# Autodesk Inventor assembly: ASY МОО 001 отстойник осветлитель
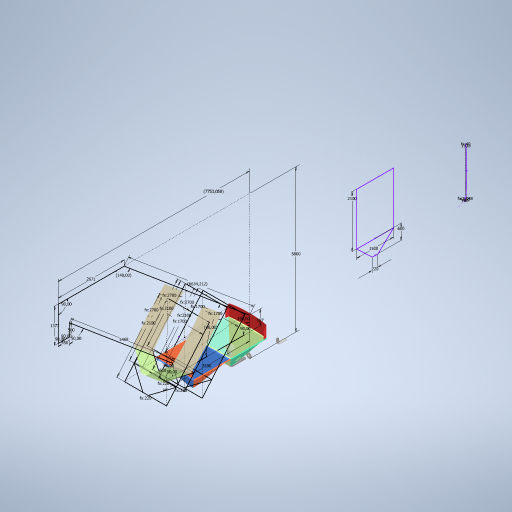
[picture p0: Inventor's stored thumbnail of the model, 512x512]
Saved by Autodesk Inventor 2024.2 (Build 282272000, 272)
## iProperties
Created: 2024-04-28
Part Number: ASY МОО 001 отстойник осветлитель
Document SubType Name: Weldment
Designer: admin
Weld Material: Welded Aluminum-6061
Mass: 420020 g
Surface Area: 719213 cm^2
Volume: 106788 cm^3
Density: 3.93322 g/cm^3
Author: admin
## Documents named in this file (20)
- C:\Users\admin\YandexDisk-badmisterfox\домашниий пк\Inventor\Manturovo\Manturovo_Se-clar\ASY МОО 001 отстойник осветлитель.iam
- C:\Users\admin\YandexDisk-badmisterfox\домашниий пк\Inventor\Manturovo\Manturovo_Se-clar\МОО 020 лист борт 1.ipt
- C:\Users\admin\YandexDisk-badmisterfox\домашниий пк\Inventor\Manturovo\Manturovo_Se-clar\МОО 010 лист спина 1.ipt
- C:\Users\admin\YandexDisk-badmisterfox\домашниий пк\Inventor\Manturovo\Manturovo_Se-clar\Пример емкости.ipt
- C:\Users\admin\YandexDisk-badmisterfox\домашниий пк\Inventor\Manturovo\Manturovo_Se-clar\МОО 030 лист брюхо 1.ipt
- C:\Users\admin\YandexDisk-badmisterfox\домашниий пк\Inventor\Manturovo\Manturovo_Se-clar\МОО 040 шпангоут борт 1.ipt
- C:\Users\admin\YandexDisk-badmisterfox\домашниий пк\Inventor\Manturovo\Manturovo_Se-clar\МОО 041 шпангоут спина 1.ipt
- C:\Users\admin\YandexDisk-badmisterfox\домашниий пк\Inventor\Manturovo\Manturovo_Se-clar\МОО 050 стрингер спина 1.ipt
- C:\Users\admin\YandexDisk-badmisterfox\домашниий пк\Inventor\Manturovo\Manturovo_Se-clar\Рама основания\ASY МОО 040 рама основания.iam
- C:\Users\admin\YandexDisk-badmisterfox\домашниий пк\Inventor\Manturovo\Manturovo_Se-clar\ASY МОО 060 ракета.iam
- C:\Users\admin\YandexDisk-badmisterfox\домашниий пк\Inventor\Manturovo\Manturovo_Se-clar\Content Center Files\en-US\ISO 5251 B 3D\ISO 5251 Bends 3D without straight ends(90 deg) DN80 2 2.ipt
- C:\Users\admin\YandexDisk-badmisterfox\домашниий пк\Inventor\Manturovo\Manturovo_Se-clar\Content Center Files\en-US\ISO 5251(1)\ISO 5251 Concentric reducers DN80 x DN65 3,2 3,2.ipt
- C:\Users\admin\YandexDisk-badmisterfox\домашниий пк\Inventor\Manturovo\Manturovo_Se-clar\ASY МОО 020 конус.iam
- C:\Users\admin\YandexDisk-badmisterfox\домашниий пк\Inventor\Manturovo\Manturovo_Se-clar\ракета\МОО 064 ракета труба.ipt
- C:\Users\admin\YandexDisk-badmisterfox\домашниий пк\Inventor\Manturovo\Manturovo_Se-clar\х_размеры МОО отстойник осветлитель Dummu.ipt
- C:\Users\admin\YandexDisk-badmisterfox\домашниий пк\Inventor\Manturovo\Manturovo_Se-clar\МОО 012 лист спина 2.ipt
- C:\Users\admin\YandexDisk-badmisterfox\домашниий пк\Inventor\Manturovo\Manturovo_Se-clar\ракета\МОО 065 ракета труба 5.ipt
- C:\Users\admin\YandexDisk-badmisterfox\домашниий пк\Inventor\Manturovo\Manturovo_Se-clar\ракета\МОО 066 ракета труба 6.ipt
- C:\Users\admin\YandexDisk-badmisterfox\домашниий пк\Inventor\Manturovo\Manturovo_Se-clar\ракета\МОО 067 ракета труба 7.ipt
- C:\Users\admin\YandexDisk-badmisterfox\домашниий пк\Inventor\Manturovo\Manturovo_Se-clar\Content Center Files\en-US\DIN EN 1092-1 01 - PN 25\DIN EN 1092-1 Plate Flange for Welding Type 01 - PN 25 80 x 88.9.ipt
## Components (52 placed, 19 different names)
1. Пример емкости:1 — Mate:1, Mate:2, Mate:3, Mate:4, Flush:2
2. х_размеры МОО отстойник осветлитель Dummu:1
3. ASY МОО 040 рама основания:1 [sub-assembly] — Flush:19, Flush:20, Flush:21
4. МОО 020 лист борт 1:2 — Flush:6, Angle:1, Symmetry:1, Mate:5, Mate:8
5. МОО 010 лист спина 1:1 — Flush:1, Mate:3, Mate:4, Flush:3, Flush:6, Mate:7, Mate:8, Mate:10
6. МОО 020 лист борт 1:1 — Flush:1, Symmetry:1, Mate:6, Flush:7, Mate:7, Mate:10, Flush:8, Flush:9, Flush:13
7. МОО 030 лист брюхо 1:1 — Mate:5, Mate:6, Flush:7, Mate:9
8. ASY МОО 060 ракета:1 [sub-assembly] — Flush:23, Rigid:10
9. ISO 5251 Bends 3D without straight ends(90 deg) DN80 2:1 — Rigid:2, Rigid:3
10. ISO 5251 Concentric reducers DN80 x DN65 3,2:1 — Rigid:2, Rigid:10
11. ASY МОО 020 конус:1 [sub-assembly] — Flush:22, Mate:16, Tangent:1, Flush:28
12. МОО 064 ракета труба:1 — Rigid:3, Cylindrical:1
13. МОО 010 лист спина 1:2
14. МОО 010 лист спина 1:3 — Flush:24
15. МОО 012 лист спина 2:1 — Mate:15, Mate:16, Tangent:1, Flush:27
16. МОО 065 ракета труба 5:1 — Rigid:5
17. МОО 066 ракета труба 6:1 — Rigid:5, Rigid:6
18. МОО 067 ракета труба 7:1 — Rigid:6, Rigid:7
19. DIN EN 1092-1 Plate Flange for Welding Type 01 - PN 25 80 x 88.9:1 — Flush:25, Flush:26, Mate:18, Cylindrical:1
20. ISO 5251 Concentric reducers DN80 x DN65 3,2:2 — Rigid:7
21. МОО 040 шпангоут борт 1:1 — Flush:8, Flush:9, Flush:10, Symmetry:2, Flush:11, Mate:11, Flush:14
22. МОО 041 шпангоут спина 1:2 — Mate:11, Flush:12
23. МОО 040 шпангоут борт 1:2 — Flush:10, Symmetry:2, Flush:11, Flush:15, Flush:16
24. МОО 040 шпангоут борт 1:3
25. МОО 041 шпангоут спина 1:3
26. МОО 040 шпангоут борт 1:4
27. МОО 040 шпангоут борт 1:5
28. МОО 041 шпангоут спина 1:4
29. МОО 040 шпангоут борт 1:6
30. МОО 040 шпангоут борт 1:7
31. МОО 041 шпангоут спина 1:5
32. МОО 040 шпангоут борт 1:8
33. МОО 040 шпангоут борт 1:9
34. МОО 041 шпангоут спина 1:6
35. МОО 040 шпангоут борт 1:10
36. МОО 040 шпангоут борт 1:11
37. МОО 041 шпангоут спина 1:7
38. МОО 040 шпангоут борт 1:12
39. МОО 040 шпангоут борт 1:13
40. МОО 041 шпангоут спина 1:8
41. МОО 040 шпангоут борт 1:14
42. МОО 040 шпангоут борт 1:15
43. МОО 041 шпангоут спина 1:9
44. МОО 040 шпангоут борт 1:16
45. МОО 050 стрингер спина 1:1 — Flush:13, Flush:14, Flush:17
46. МОО 050 стрингер спина 1:2 — Flush:15, Flush:16, Flush:17
47. МОО 050 стрингер спина 1:3
48. МОО 050 стрингер спина 1:4
49. МОО 050 стрингер спина 1:5
50. МОО 050 стрингер спина 1:6
51. МОО 050 стрингер спина 1:7
52. МОО 050 стрингер спина 1:8
## Component patterns: (8 elements, first: МОО 040 шпангоут борт 1:1 + МОО 041 шпангоут спина 1:2 + МОО 040 шпангоут борт 1:2), (4 elements, first: МОО 050 стрингер спина 1:1 + МОО 050 стрингер спина 1:2)
## Relationships (50: Flush 25, Mate 14, WeldJoint 6, Symmetry 2, Angle 1, Tangent 1, CylindricalJoint 1)
- Flush:1: МОО 010 лист спина 1:1 ↔ МОО 020 лист борт 1:1
- Mate:1: Пример емкости:1
- Mate:2: Пример емкости:1
- Mate:3: Пример емкости:1 ↔ МОО 010 лист спина 1:1
- Mate:4: Пример емкости:1 ↔ МОО 010 лист спина 1:1
- Flush:2: Пример емкости:1
- Flush:3: МОО 010 лист спина 1:1
- Flush:6: МОО 020 лист борт 1:2 ↔ МОО 010 лист спина 1:1
- Angle:1 (180 deg): МОО 020 лист борт 1:2
- Symmetry:1: МОО 020 лист борт 1:2 ↔ МОО 020 лист борт 1:1
- Mate:5: МОО 020 лист борт 1:2 ↔ МОО 030 лист брюхо 1:1
- Mate:6: МОО 020 лист борт 1:1 ↔ МОО 030 лист брюхо 1:1
- Flush:7: МОО 020 лист борт 1:1 ↔ МОО 030 лист брюхо 1:1
- Mate:7: МОО 010 лист спина 1:1 ↔ МОО 020 лист борт 1:1
- Mate:8: МОО 020 лист борт 1:2 ↔ МОО 010 лист спина 1:1
- Mate:9: МОО 030 лист брюхо 1:1
- Mate:10 (-20 mm): МОО 010 лист спина 1:1 ↔ МОО 020 лист борт 1:1
- Flush:8: МОО 020 лист борт 1:1 ↔ МОО 040 шпангоут борт 1:1
- Flush:9 (250 mm): МОО 020 лист борт 1:1 ↔ МОО 040 шпангоут борт 1:1
- Flush:10: МОО 040 шпангоут борт 1:1 ↔ МОО 040 шпангоут борт 1:2
- Symmetry:2: МОО 040 шпангоут борт 1:1 ↔ МОО 040 шпангоут борт 1:2
- Flush:11: МОО 040 шпангоут борт 1:1 ↔ МОО 040 шпангоут борт 1:2
- Mate:11: МОО 040 шпангоут борт 1:1 ↔ МОО 041 шпангоут спина 1:2
- Flush:12: МОО 041 шпангоут спина 1:2
- Flush:13: МОО 020 лист борт 1:1 ↔ МОО 050 стрингер спина 1:1
- Flush:14 (3 mm): МОО 040 шпангоут борт 1:1 ↔ МОО 050 стрингер спина 1:1
- Flush:15 (-250 mm): МОО 040 шпангоут борт 1:2 ↔ МОО 050 стрингер спина 1:2
- Flush:16 (3 mm): МОО 040 шпангоут борт 1:2 ↔ МОО 050 стрингер спина 1:2
- Flush:17: МОО 050 стрингер спина 1:1 ↔ МОО 050 стрингер спина 1:2
- Rigid:2 [WeldJoint]: ISO 5251 Bends 3D without straight ends(90 deg) DN80 2:1 ↔ ISO 5251 Concentric reducers DN80 x DN65 3,2:1
- Rigid:3 [WeldJoint]: ISO 5251 Bends 3D without straight ends(90 deg) DN80 2:1 ↔ МОО 064 ракета труба:1
- Flush:19 (-250 mm): ASY МОО 040 рама основания:1
- Flush:20: ASY МОО 040 рама основания:1
- Flush:21: ASY МОО 040 рама основания:1
- Flush:22: ASY МОО 020 конус:1
- Flush:23: ASY МОО 060 ракета:1
- Mate:15: МОО 012 лист спина 2:1
- Flush:24: МОО 010 лист спина 1:3
- Mate:16: ASY МОО 020 конус:1 ↔ МОО 012 лист спина 2:1
- Tangent:1 (-5 mm): ASY МОО 020 конус:1 ↔ МОО 012 лист спина 2:1
- Rigid:5 [WeldJoint]: МОО 065 ракета труба 5:1 ↔ МОО 066 ракета труба 6:1
- Rigid:6 [WeldJoint]: МОО 066 ракета труба 6:1 ↔ МОО 067 ракета труба 7:1
- Flush:25: DIN EN 1092-1 Plate Flange for Welding Type 01 - PN 25 80 x 88.9:1
- Flush:26: DIN EN 1092-1 Plate Flange for Welding Type 01 - PN 25 80 x 88.9:1
- Mate:18 (120 mm): DIN EN 1092-1 Plate Flange for Welding Type 01 - PN 25 80 x 88.9:1
- Rigid:7 [WeldJoint]: МОО 067 ракета труба 7:1 ↔ ISO 5251 Concentric reducers DN80 x DN65 3,2:2
- Rigid:10 [WeldJoint] (-20 mm): ASY МОО 060 ракета:1 ↔ ISO 5251 Concentric reducers DN80 x DN65 3,2:1
- Cylindrical:1: МОО 064 ракета труба:1 ↔ DIN EN 1092-1 Plate Flange for Welding Type 01 - PN 25 80 x 88.9:1
- Flush:27 (40 mm): МОО 012 лист спина 2:1
- Flush:28: ASY МОО 020 конус:1
